# Autodesk Inventor assembly: bomba_hidraulica
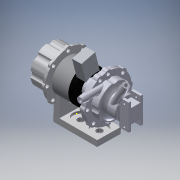
[picture p0: Inventor's stored thumbnail of the model, 180x180]
Saved by Autodesk Inventor 2019 (Build 230136000, 136)
## iProperties
Created: 2019-09-28
Part Number: bomba_hidraulica
Document SubType Name: Assembly
Designer: dbrau
Author: dbrau
## Documents named in this file (6)
- D:\U\Semestre III mecánica\seminario\bomba_hidraulica.iam
- D:\U\Semestre III mecánica\seminario\motor_hidraulica.ipt
- D:\U\Semestre III mecánica\seminario\tapa inferior.ipt
- D:\U\Semestre III mecánica\seminario\tapa turbina.ipt
- D:\U\Semestre III mecánica\seminario\topa_motor.ipt
- D:\U\Semestre III mecánica\seminario\turbina.ipt
## Components (5 placed, 5 different names)
1. motor_hidraulica:1 — Insert:1, Insert:2
2. tapa turbina:1 — Insert:4, Insert:5
3. topa_motor:1 — Insert:1
4. tapa inferior:1 — Insert:2, Insert:3, Insert:4, Insert:5
5. turbina:1 — Insert:3
## Relationships (5: Insert 5)
- Insert:1: motor_hidraulica:1 ↔ topa_motor:1
- Insert:2: motor_hidraulica:1 ↔ tapa inferior:1
- Insert:3: tapa inferior:1 ↔ turbina:1
- Insert:4: tapa turbina:1 ↔ tapa inferior:1
- Insert:5: tapa turbina:1 ↔ tapa inferior:1
